# Autodesk Inventor assembly: forward_assembly
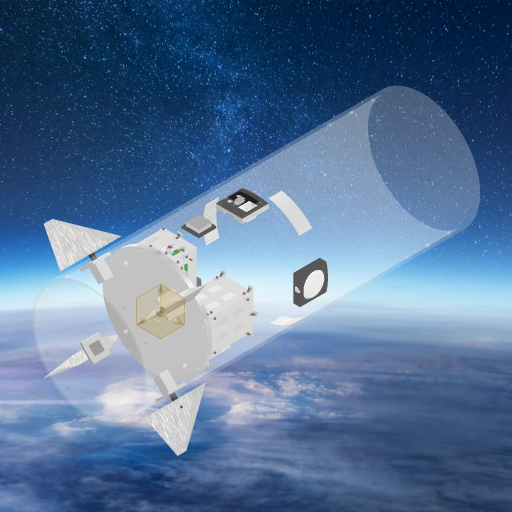
[picture p0: Inventor's stored thumbnail of the model, 512x512]
Saved by Autodesk Inventor 2023 (Build 270158000, 158)
## iProperties
Created: 2023-03-23
Part Number: forward_assembly
Document SubType Name: Assembly
Designer: 310611102
Mass: 9762.82 g
Surface Area: 17061.5 cm^2
Volume: 3787.99 cm^3
Density: 2.57731 g/cm^3
Author: 310611102
## Documents named in this file (31)
- C:\Users\310611102\Documents\Inventor\SSR\avionics_2023ver\assembly\forward_assembly.iam
- C:\Users\310611102\Documents\Inventor\SSR\avionics_2023ver\assembly\Tube - Forward Section.ipt
- C:\Users\310611102\Documents\Inventor\SSR\avionics_2023ver\actuator_system\actuator_system.iam
- C:\Users\310611102\Documents\Inventor\SSR\avionics_2023ver\electronics\patch_antenna.ipt
- C:\Users\310611102\Documents\Inventor\SSR\avionics_2023ver\electronics\battery_24V.ipt
- C:\Users\310611102\Documents\Inventor\SSR\avionics_2023ver\electronics\battery box\battery_box_ver3\battery_box_24V.iam
- C:\Users\310611102\Documents\Inventor\SSR\avionics_2023ver\electronics\battery_5V.ipt
- C:\Users\310611102\Documents\Inventor\SSR\avionics_2023ver\electronics\battery box2\battery_box_5V_ver2\battery_box_5V.iam
- C:\Users\310611102\Documents\Inventor\SSR\avionics_2023ver\actuator_system\Forward_lower plate.ipt
- C:\Users\310611102\Documents\Inventor\SSR\avionics_2023ver\actuator_system\gearbox_temp\coupling.ipt
- C:\Users\310611102\Documents\Inventor\SSR\avionics_2023ver\electronics\socket_assembly.iam
- C:\Users\310611102\Documents\Inventor\SSR\avionics_2023ver\electronics\antenna_socket.ipt
- C:\Users\310611102\Documents\Inventor\SSR\avionics_2023ver\electronics\GPSR_antenna.ipt
- C:\Users\310611102\Documents\Inventor\SSR\avionics_2023ver\assembly\forward_assembly\AIP\Cable and Harness\forward_assembly.Harness5.iam
- C:\Users\310611102\Documents\Inventor\SSR\avionics_2023ver\assembly\forward_assembly\AIP\Cable and Harness\forward_assembly.Harness6.iam
- C:\Users\310611102\Documents\Inventor\SSR\avionics_2023ver\assembly\forward_assembly\AIP\Cable and Harness\forward_assembly.Harness7.iam
- C:\Users\310611102\Documents\Inventor\SSR\avionics_2023ver\assembly\forward_assembly\AIP\Cable and Harness\forward_assembly.Harness8.iam
- C:\Users\310611102\Documents\Inventor\SSR\avionics_2023ver\assembly\forward_assembly\AIP\Tube and Pipe\forward_assembly.Tube and Pipe Runs4.iam
- C:\Users\310611102\Documents\Inventor\SSR\avionics_2023ver\assembly\forward_assembly\AIP\Cable and Harness\forward_assembly.Harness11.iam
- C:\Users\310611102\Documents\Inventor\SSR\avionics_2023ver\assembly\pad.ipt
- C:\Users\310611102\Documents\Inventor\SSR\avionics_2023ver\actuator_system\gearbox_temp\gearbox_temp.iam
- C:\Users\310611102\Documents\Inventor\SSR\avionics_2023ver\electronics\antenna_socket_cap.ipt
- C:\Users\310611102\Documents\Inventor\SSR\avionics_2023ver\assembly\Fiberglass tube 0.75m.ipt
- C:\Users\310611102\Documents\Inventor\SSR\avionics_2023ver\assembly\canard_assemb.iam
- C:\Users\310611102\Documents\Inventor\SSR\avionics_2023ver\assembly\PA_assemb.iam
- C:\Users\310611102\Documents\Inventor\SSR\avionics_2023ver\assembly\cooler_plate_assemb.iam
- C:\Users\310611102\Documents\Inventor\SSR\avionics_2023ver\assembly\avionics_reassemb.iam
- C:\Users\310611102\Documents\Inventor\SSR\avionics_2023ver\assembly\canard_assemb2.iam
- C:\Users\310611102\Documents\Inventor\SSR\avionics_2023ver\assembly\canard_assemb3.iam
- C:\Users\310611102\Documents\Inventor\SSR\avionics_2023ver\assembly\antenna_assemb.iam
- C:\Users\310611102\Documents\Inventor\SSR\avionics_2023ver\assembly\Fiberglass tube 0.75m(1).ipt
## Components (43 placed, 30 different names)
1. Fiberglass tube 0.75m(1):1 — Mate:25, Flush:40
2. Fiberglass tube 0.75m:1 — Cylindrical:21, Cylindrical:23, Cylindrical:24, Cylindrical:25, Flush:39, Angle:6, Mate:23, Mate:24, Cylindrical:26, Cylindrical:27, Cylindrical:28, Cylindrical:29, Mate:25, Flush:40
3. Tube - Forward Section:1 — Cylindrical:2, Mate:5, Mate:6, Mate:7, Cylindrical:5, Cylindrical:6, Mate:21
4. actuator_system:1 [sub-assembly] — Cylindrical:2, Mate:7, Angle:1, Insert:47
5. battery_24V:1 — Mate:10, Mate:11, Mate:12
6. battery_box_24V:1 [sub-assembly] — Mate:10, Mate:11, Mate:12, Angle:1, Insert:50, Insert:53, Mate:19, Flush:2, Flush:3
7. battery_5V:1 — Mate:13, Mate:15
8. battery_box_5V:1 [sub-assembly] — Mate:13, Mate:15, Insert:48, Insert:49
9. Forward_lower plate:1 — Cylindrical:5, Insert:47, Insert:48, Insert:49, Insert:50, Insert:53, Mate:22, Insert:84, Insert:97, Cylindrical:21, Flush:39, Insert:137, Insert:138, Insert:139, Insert:140, Insert:141, Insert:142
10. socket_assembly:1 [sub-assembly] — Angle:5, Cylindrical:23
11. Harness5 [sub-assembly]
12. Harness6 [sub-assembly]
13. Harness7 [sub-assembly]
14. Harness8 [sub-assembly]
15. Tube & Pipe Runs4 [sub-assembly]
16. Harness11 [sub-assembly]
17. pad:1 — Mate:19, Flush:2, Flush:3
18. gearbox_temp:1 [sub-assembly] — Mate:22, Insert:84, Insert:97, Insert:98
19. coupling:1 — Insert:98
20. GPSR_antenna:1 — Insert:136
21. antenna_socket:1 — Angle:2, Mate:21, Insert:99, Insert:100, Insert:136
22. antenna_socket_cap:1 — Insert:99, Insert:100
23. PA_assemb:1 [sub-assembly] — Insert:137, Insert:138
24. cooler_plate_assemb:1 [sub-assembly] — Mate:23, Mate:24
25. avionics_reassemb:1 [sub-assembly] — Insert:139, Insert:140
26. patch_antenna:1 — Cylindrical:6, Angle:3
27. patch_antenna:2
28. patch_antenna:3
29. canard_assemb:1 [sub-assembly] — Cylindrical:24, Cylindrical:25
30. canard_assemb:2 [sub-assembly]
31. canard_assemb:3 [sub-assembly]
32. canard_assemb:4 [sub-assembly]
33. canard_assemb2:1 [sub-assembly] — Cylindrical:26, Cylindrical:27
34. canard_assemb2:2 [sub-assembly]
35. canard_assemb2:3 [sub-assembly]
36. canard_assemb2:4 [sub-assembly]
37. canard_assemb3:1 [sub-assembly] — Cylindrical:28, Cylindrical:29
38. canard_assemb3:2 [sub-assembly]
39. canard_assemb3:3 [sub-assembly]
40. canard_assemb3:4 [sub-assembly]
41. antenna_assemb:1 [sub-assembly] — Insert:141, Insert:142
42. antenna_assemb:2 [sub-assembly]
43. antenna_assemb:3 [sub-assembly]
## Component patterns: (3 elements, first: patch_antenna:1), Canard_pattern1 (4 elements), Canard_pattern2 (4 elements), Canard_pattern3 (4 elements), (3 elements, first: antenna_assemb:1)
## Relationships (51: Insert 17, Mate 14, CylindricalJoint 11, Angle 5, Flush 4)
- Cylindrical:2: Tube - Forward Section:1 ↔ actuator_system:1
- Mate:5: Tube - Forward Section:1
- Mate:6: Tube - Forward Section:1
- Mate:7: Tube - Forward Section:1 ↔ actuator_system:1
- Mate:10: battery_24V:1 ↔ battery_box_24V:1
- Mate:11: battery_24V:1 ↔ battery_box_24V:1
- Mate:12: battery_24V:1 ↔ battery_box_24V:1
- Angle:1 (0 deg): actuator_system:1 ↔ battery_box_24V:1
- Mate:13: battery_5V:1 ↔ battery_box_5V:1
- Mate:15: battery_5V:1 ↔ battery_box_5V:1
- Cylindrical:5: Tube - Forward Section:1 ↔ Forward_lower plate:1
- Insert:47: actuator_system:1 ↔ Forward_lower plate:1
- Insert:48: battery_box_5V:1 ↔ Forward_lower plate:1
- Insert:49: battery_box_5V:1 ↔ Forward_lower plate:1
- Insert:50: battery_box_24V:1 ↔ Forward_lower plate:1
- Insert:53: battery_box_24V:1 ↔ Forward_lower plate:1
- Cylindrical:6: Tube - Forward Section:1 ↔ patch_antenna:1
- Angle:2 (270 deg): antenna_socket:1
- Angle:3 (102 deg): patch_antenna:1
- Angle:5 (180 deg): socket_assembly:1
- Mate:19: battery_box_24V:1 ↔ pad:1
- Flush:2: battery_box_24V:1 ↔ pad:1
- Flush:3: battery_box_24V:1 ↔ pad:1
- Mate:21 (50 mm): Tube - Forward Section:1 ↔ antenna_socket:1
- Mate:22: Forward_lower plate:1 ↔ gearbox_temp:1
- Insert:84: Forward_lower plate:1 ↔ gearbox_temp:1
- Insert:97: Forward_lower plate:1 ↔ gearbox_temp:1
- Insert:98: gearbox_temp:1 ↔ coupling:1
- Insert:99: antenna_socket:1 ↔ antenna_socket_cap:1
- Insert:100: antenna_socket:1 ↔ antenna_socket_cap:1
- Cylindrical:21: Fiberglass tube 0.75m:1 ↔ Forward_lower plate:1
- Cylindrical:23: Fiberglass tube 0.75m:1 ↔ socket_assembly:1
- Insert:136: GPSR_antenna:1 ↔ antenna_socket:1
- Cylindrical:24: Fiberglass tube 0.75m:1 ↔ canard_assemb:1
- Cylindrical:25: Fiberglass tube 0.75m:1 ↔ canard_assemb:1
- Flush:39 (150 mm): Fiberglass tube 0.75m:1 ↔ Forward_lower plate:1
- Angle:6 (0 deg): Fiberglass tube 0.75m:1
- Insert:137: Forward_lower plate:1 ↔ PA_assemb:1
- Insert:138: Forward_lower plate:1 ↔ PA_assemb:1
- Mate:23: Fiberglass tube 0.75m:1 ↔ cooler_plate_assemb:1
- Mate:24: Fiberglass tube 0.75m:1 ↔ cooler_plate_assemb:1
- Insert:139: Forward_lower plate:1 ↔ avionics_reassemb:1
- Insert:140: Forward_lower plate:1 ↔ avionics_reassemb:1
- Cylindrical:26: Fiberglass tube 0.75m:1 ↔ canard_assemb2:1
- Cylindrical:27: Fiberglass tube 0.75m:1 ↔ canard_assemb2:1
- Cylindrical:28: Fiberglass tube 0.75m:1 ↔ canard_assemb3:1
- Cylindrical:29: Fiberglass tube 0.75m:1 ↔ canard_assemb3:1
- Insert:141: Forward_lower plate:1 ↔ antenna_assemb:1
- Insert:142: Forward_lower plate:1 ↔ antenna_assemb:1
- Mate:25: Fiberglass tube 0.75m(1):1 ↔ Fiberglass tube 0.75m:1
- Flush:40: Fiberglass tube 0.75m(1):1 ↔ Fiberglass tube 0.75m:1
